# Autodesk Inventor assembly: oled-2.42-variant
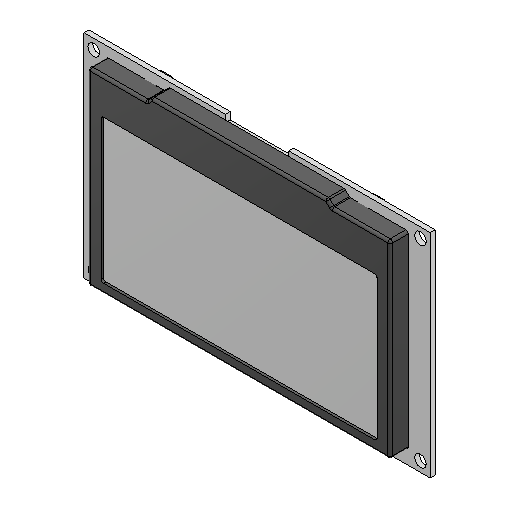
[picture p0: Inventor's stored thumbnail of the model, 512x512]
Saved by Autodesk Inventor 2026 (Build 300175050, 175E)
## iProperties
Created: 2025-06-21
Part Number: oled-2.42-variant
Document SubType Name: Assembly
Designer: queezz
Author: queezz
## Documents named in this file (3)
- C:\Users\queezz\Dropbox\Drawings\PIHTI\ElectronicsBox\esp32-ambient-logger\oled-2.42-variant.iam
- C:\Users\queezz\Dropbox\Drawings\PIHTI\ElectronicsBox\esp32-ambient-logger\oled2.42-pcb.ipt
- C:\Users\queezz\Dropbox\Drawings\PIHTI\ElectronicsBox\esp32-ambient-logger\STEPs\OLED 2.42 12864 v7\screen.ipt
## Components (2 placed, 2 different names)
1. oled2.42-pcb:1 — Mate:1, Flush:1, Flush:2
2. screen:1 — Mate:1, Flush:1, Flush:2
## Relationships (3: Flush 2, Mate 1)
- Mate:1: oled2.42-pcb:1 ↔ screen:1
- Flush:1 (1 mm): oled2.42-pcb:1 ↔ screen:1
- Flush:2 (4.5 mm): oled2.42-pcb:1 ↔ screen:1
